# Autodesk Inventor assembly: UpperArm
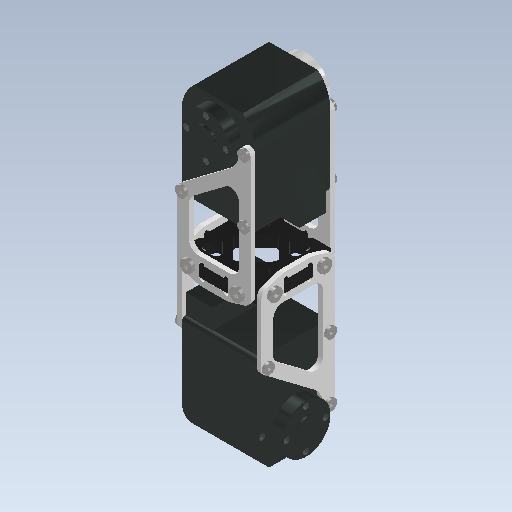
[picture p0: Inventor's stored thumbnail of the model, 512x512]
Saved by Autodesk Inventor 2020.4 (Build 244396000, 396)
## iProperties
Created: 2021-09-11
Part Number: UpperArm
Document SubType Name: Assembly
Designer: Masato
Author: Masato
## Documents named in this file (8)
- C:\Users\Masato\Documents\Inventor\CIT Brains_Inventor\OpenPlatform_ver3_0\UpperBody\Arm\UpperArm.iam
- C:\Users\Masato\Documents\Inventor\CIT Brains_Inventor\OpenPlatform_ver3_0\UpperBody\Arm\UpperArm_vertical_frame_01.ipt
- C:\Users\Masato\Documents\Inventor\CIT Brains_Inventor\OpenPlatform_ver3_0\UpperBody\Arm\UpperArm_horizontal_frame_01.ipt
- C:\Users\Masato\Documents\Inventor\CIT Brains_Inventor\OpenPlatform_ver3_0\Ready_Made\B3M10xx.ipt
- C:\Users\Masato\Documents\Inventor\CIT Brains_Inventor\OpenPlatform_ver3_0\Ready_Made\free_horn.ipt
- C:\Users\Masato\Documents\Inventor\CIT Brains_Inventor\OpenPlatform_ver3_0\Ready_Made\Screw\M2_6-15.ipt
- C:\Users\Masato\Documents\Inventor\CIT Brains_Inventor\OpenPlatform_ver3_0\Ready_Made\Screw\M2_6-20.ipt
- C:\Users\Masato\Documents\Inventor\CIT Brains_Inventor\OpenPlatform_ver3_0\Ready_Made\Screw\M3-6.ipt
## Components (29 placed, 7 different names)
1. UpperArm_horizontal_frame_01:1 — 挿入:7, 挿入:8, 挿入:9, 挿入:10, 挿入:11, 挿入:12, 挿入:13, 挿入:14
2. UpperArm_vertical_frame_01:1 — 挿入:1, 挿入:2, 挿入:3, 挿入:7, 挿入:8, 挿入:29, 挿入:30, 挿入:31, 挿入:37, 挿入:38
3. UpperArm_vertical_frame_01:2 — 挿入:4, 挿入:5, 挿入:6, 挿入:9, 挿入:10, 挿入:23, 挿入:24, 挿入:25, 挿入:41, 挿入:42
4. UpperArm_vertical_frame_01:3 — 挿入:11, 挿入:12, 挿入:15, 挿入:16, 挿入:17, 挿入:26, 挿入:27, 挿入:28, 挿入:39, 挿入:40
5. UpperArm_vertical_frame_01:4 — 挿入:13, 挿入:14, 挿入:18, 挿入:19, 挿入:20, 挿入:32, 挿入:33, 挿入:34, 挿入:35, 挿入:36
6. B3M10xx:1 — 挿入:1, 挿入:2, 挿入:3, 挿入:4, 挿入:5, 挿入:6, 挿入:22
7. B3M10xx:2 — 挿入:15, 挿入:16, 挿入:17, 挿入:18, 挿入:19, 挿入:20, 挿入:21
8. free_horn:1 — 挿入:22
9. free_horn:2 — 挿入:21
10. M2_6-15:1 — 挿入:23
11. M2_6-15:2 — 挿入:24
12. M2_6-15:3 — 挿入:25
13. M2_6-15:4 — 挿入:26
14. M2_6-15:5 — 挿入:27
15. M2_6-15:6 — 挿入:28
16. M2_6-20:1 — 挿入:29
17. M2_6-20:2 — 挿入:30
18. M2_6-20:3 — 挿入:31
19. M2_6-20:4 — 挿入:32
20. M2_6-20:5 — 挿入:33
21. M2_6-20:6 — 挿入:34
22. M3-6:1 — 挿入:35
23. M3-6:2 — 挿入:36
24. M3-6:3 — 挿入:37
25. M3-6:4 — 挿入:38
26. M3-6:5 — 挿入:39
27. M3-6:6 — 挿入:40
28. M3-6:7 — 挿入:41
29. M3-6:8 — 挿入:42
## Relationships (42: Insert 42)
- 挿入:1 [Insert]: UpperArm_vertical_frame_01:1 ↔ B3M10xx:1
- 挿入:2 [Insert]: UpperArm_vertical_frame_01:1 ↔ B3M10xx:1
- 挿入:3 [Insert]: UpperArm_vertical_frame_01:1 ↔ B3M10xx:1
- 挿入:4 [Insert]: UpperArm_vertical_frame_01:2 ↔ B3M10xx:1
- 挿入:5 [Insert]: UpperArm_vertical_frame_01:2 ↔ B3M10xx:1
- 挿入:6 [Insert]: UpperArm_vertical_frame_01:2 ↔ B3M10xx:1
- 挿入:7 [Insert]: UpperArm_horizontal_frame_01:1 ↔ UpperArm_vertical_frame_01:1
- 挿入:8 [Insert]: UpperArm_horizontal_frame_01:1 ↔ UpperArm_vertical_frame_01:1
- 挿入:9 [Insert]: UpperArm_horizontal_frame_01:1 ↔ UpperArm_vertical_frame_01:2
- 挿入:10 [Insert]: UpperArm_horizontal_frame_01:1 ↔ UpperArm_vertical_frame_01:2
- 挿入:11 [Insert]: UpperArm_horizontal_frame_01:1 ↔ UpperArm_vertical_frame_01:3
- 挿入:12 [Insert]: UpperArm_horizontal_frame_01:1 ↔ UpperArm_vertical_frame_01:3
- 挿入:13 [Insert]: UpperArm_horizontal_frame_01:1 ↔ UpperArm_vertical_frame_01:4
- 挿入:14 [Insert]: UpperArm_horizontal_frame_01:1 ↔ UpperArm_vertical_frame_01:4
- 挿入:15 [Insert]: UpperArm_vertical_frame_01:3 ↔ B3M10xx:2
- 挿入:16 [Insert]: UpperArm_vertical_frame_01:3 ↔ B3M10xx:2
- 挿入:17 [Insert]: UpperArm_vertical_frame_01:3 ↔ B3M10xx:2
- 挿入:18 [Insert]: UpperArm_vertical_frame_01:4 ↔ B3M10xx:2
- 挿入:19 [Insert]: UpperArm_vertical_frame_01:4 ↔ B3M10xx:2
- 挿入:20 [Insert]: UpperArm_vertical_frame_01:4 ↔ B3M10xx:2
- 挿入:21 [Insert]: B3M10xx:2 ↔ free_horn:2
- 挿入:22 [Insert]: B3M10xx:1 ↔ free_horn:1
- 挿入:23 [Insert]: UpperArm_vertical_frame_01:2 ↔ M2_6-15:1
- 挿入:24 [Insert]: UpperArm_vertical_frame_01:2 ↔ M2_6-15:2
- 挿入:25 [Insert]: UpperArm_vertical_frame_01:2 ↔ M2_6-15:3
- 挿入:26 [Insert]: UpperArm_vertical_frame_01:3 ↔ M2_6-15:4
- 挿入:27 [Insert]: UpperArm_vertical_frame_01:3 ↔ M2_6-15:5
- 挿入:28 [Insert]: UpperArm_vertical_frame_01:3 ↔ M2_6-15:6
- 挿入:29 [Insert]: UpperArm_vertical_frame_01:1 ↔ M2_6-20:1
- 挿入:30 [Insert]: UpperArm_vertical_frame_01:1 ↔ M2_6-20:2
- 挿入:31 [Insert]: UpperArm_vertical_frame_01:1 ↔ M2_6-20:3
- 挿入:32 [Insert]: UpperArm_vertical_frame_01:4 ↔ M2_6-20:4
- 挿入:33 [Insert]: UpperArm_vertical_frame_01:4 ↔ M2_6-20:5
- 挿入:34 [Insert]: UpperArm_vertical_frame_01:4 ↔ M2_6-20:6
- 挿入:35 [Insert]: UpperArm_vertical_frame_01:4 ↔ M3-6:1
- 挿入:36 [Insert]: UpperArm_vertical_frame_01:4 ↔ M3-6:2
- 挿入:37 [Insert]: UpperArm_vertical_frame_01:1 ↔ M3-6:3
- 挿入:38 [Insert]: UpperArm_vertical_frame_01:1 ↔ M3-6:4
- 挿入:39 [Insert]: UpperArm_vertical_frame_01:3 ↔ M3-6:5
- 挿入:40 [Insert]: UpperArm_vertical_frame_01:3 ↔ M3-6:6
- 挿入:41 [Insert]: UpperArm_vertical_frame_01:2 ↔ M3-6:7
- 挿入:42 [Insert]: UpperArm_vertical_frame_01:2 ↔ M3-6:8
